# Autodesk Inventor assembly: bushing_asm
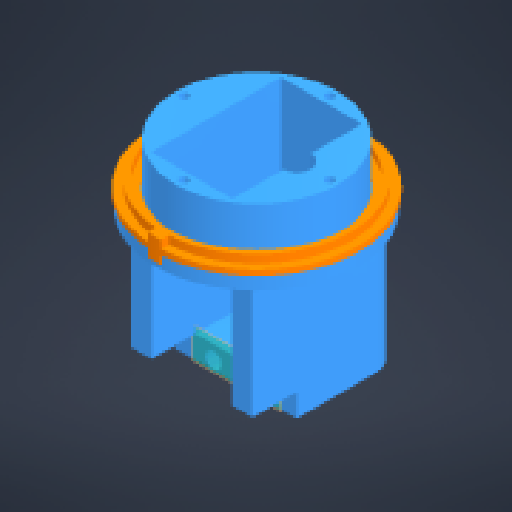
[picture p0: Inventor's stored thumbnail of the model, 512x512]
Saved by Autodesk Inventor 2024 (Build 280153000, 153)
## iProperties
Created: 2023-11-08
Part Number: bushing_asm
Document SubType Name: Assembly
Designer: user
Author: user
## Documents named in this file (3)
- D:\DOC\robot\screw_driver\3d_v2\machine_body\manipulator\bushing_asm.iam
- D:\DOC\robot\screw_driver\3d_v2\machine_body\manipulator\bushing.ipt
- D:\DOC\robot\screw_driver\3d_v2\machine_body\manipulator\ring.ipt
## Components (3 placed, 2 different names)
1. bushing:1 — Совмещение:1, Совмещение:2, Совмещение:3, Совмещение:4, Вставка:1, Угол:1, Вставка:2, Совмещение:5
2. ring:1 — Совмещение:4, Вставка:1, Угол:1
3. ring:2 — Вставка:2, Совмещение:5
## Relationships (8: Mate 5, Insert 2, Angle 1)
- Совмещение:1 [Mate]: bushing:1
- Совмещение:2 [Mate]: bushing:1
- Совмещение:3 [Mate]: bushing:1
- Совмещение:4 [Mate]: bushing:1 ↔ ring:1
- Вставка:1 [Insert]: bushing:1 ↔ ring:1
- Угол:1 [Angle] (180 deg): bushing:1 ↔ ring:1
- Вставка:2 [Insert]: bushing:1 ↔ ring:2
- Совмещение:5 [Mate]: bushing:1 ↔ ring:2
